# Autodesk Inventor assembly: BackUpperLink
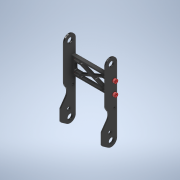
[picture p0: Inventor's stored thumbnail of the model, 180x180]
Saved by Autodesk Inventor 2022 (Build 260153000, 153)
## iProperties
Created: 2022-06-15
Part Number: BackUpperLink
Document SubType Name: Assembly
Designer: Masato Kubotera
Author: Masato Kubotera
## Documents named in this file (4)
- C:\Users\MasatoKubotera\Documents\Inventor\SUSTAINA-OP\LowerBody\Link\BackUpperLink.iam
- C:\Users\MasatoKubotera\Documents\Inventor\SUSTAINA-OP\LowerBody\Link\BackLink_diagonal.ipt
- C:\Users\MasatoKubotera\Documents\Inventor\SUSTAINA-OP\LowerBody\Link\BackLink_frame.ipt
- C:\Users\MasatoKubotera\Documents\Inventor\SUSTAINA-OP\ReadyMade\Screw\UC-0306.ipt
## Components (7 placed, 3 different names)
1. BackLink_diagonal:1 — 挿入:1, 挿入:2, 挿入:3, 挿入:4
2. BackLink_frame:1 — 挿入:1, 挿入:2, 挿入:5, 挿入:6, メイト:1, メイト:2, 対称度:1
3. BackLink_frame:2 — 挿入:3, 挿入:4, 挿入:7, 挿入:8, 対称度:1
4. UC-0306:1 — 挿入:5
5. UC-0306:2 — 挿入:6
6. UC-0306:3 — 挿入:7
7. UC-0306:4 — 挿入:8
## Relationships (16: Insert 8, Mate 7, Symmetry 1)
- 挿入:1 [Insert]: BackLink_diagonal:1 ↔ BackLink_frame:1
- 挿入:2 [Insert]: BackLink_diagonal:1 ↔ BackLink_frame:1
- 挿入:3 [Insert]: BackLink_diagonal:1 ↔ BackLink_frame:2
- 挿入:4 [Insert]: BackLink_diagonal:1 ↔ BackLink_frame:2
- 挿入:5 [Insert]: BackLink_frame:1 ↔ UC-0306:1
- 挿入:6 [Insert]: BackLink_frame:1 ↔ UC-0306:2
- 挿入:7 [Insert]: BackLink_frame:2 ↔ UC-0306:3
- 挿入:8 [Insert]: BackLink_frame:2 ↔ UC-0306:4
- メイト:1 [Mate]: BackLink_frame:1
- メイト:2 [Mate]: BackLink_frame:1
- メイト:3 [Mate]
- メイト:4 [Mate]
- メイト:5 [Mate]
- 対称度:1 [Symmetry]: BackLink_frame:1 ↔ BackLink_frame:2
- メイト:6 [Mate]
- メイト:7 [Mate]
